# Autodesk Inventor assembly: winchAssembly
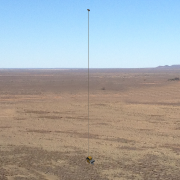
[picture p0: Inventor's stored thumbnail of the model, 180x180]
Saved by Autodesk Inventor 2013 SP2 (Build 170200200, 200)
## iProperties
Company: HERA Project
Created: 2013-12-16
Part Number: winchAssembly
Document SubType Name: Assembly
Designer: Dave
Author: David DeBoer
Title: Winch
## Documents named in this file (5)
- C:\Users\Dave\Desktop\hera-cad\support\winchAssembly.iam
- C:\Users\Dave\Desktop\hera-cad\smallParts\winch.ipt
- C:\Users\Dave\Desktop\hera-cad\support\kevlarDown.ipt
- C:\Users\Dave\Desktop\hera-cad\smallParts\thickRightAngle.ipt
- C:\Users\Dave\Desktop\hera-cad\smallParts\pulley.ipt
## Components (4 placed, 4 different names)
1. winch:1 — Insert:1
2. kevlarDown:1
3. thickRightAngle:1 — Insert:1
4. pulley:1
## Relationships (1: Insert 1)
- Insert:1: winch:1 ↔ thickRightAngle:1
